# Autodesk Inventor assembly: Lower_Arm_ConnectorJe19
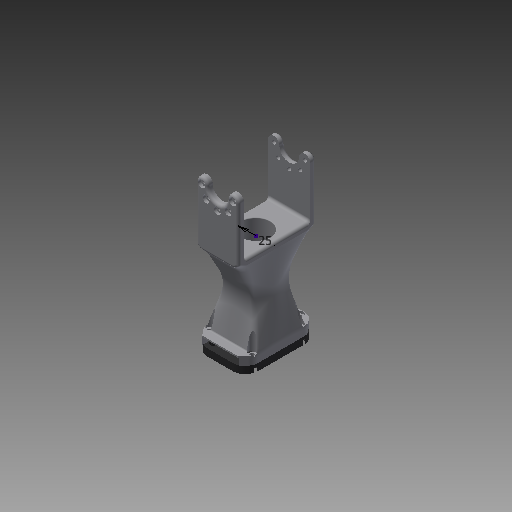
[picture p0: Inventor's stored thumbnail of the model, 512x512]
Saved by Autodesk Inventor 2019 (Build 230136000, 136)
## iProperties
Created: 2019-06-24
Part Number: Lower_Arm_ConnectorJe19
Document SubType Name: Assembly
Designer: xwermter
Author: xwermter
## Documents named in this file (3)
- Z:\nico\arms\Lower_Arm_ConnectorJe19.iam
- Z:\nico\arms\lower_arm_thick.ipt
- Z:\nico\arms\connector.ipt
## Components (2 placed, 2 different names)
1. lower_arm_thick:1 — Mate:1, Mate:2
2. connector:1 — Mate:1, Mate:2
## Relationships (2: Mate 2)
- Mate:1: lower_arm_thick:1 ↔ connector:1
- Mate:2: lower_arm_thick:1 ↔ connector:1
